# Autodesk Inventor assembly: Irradiation Fixture V1
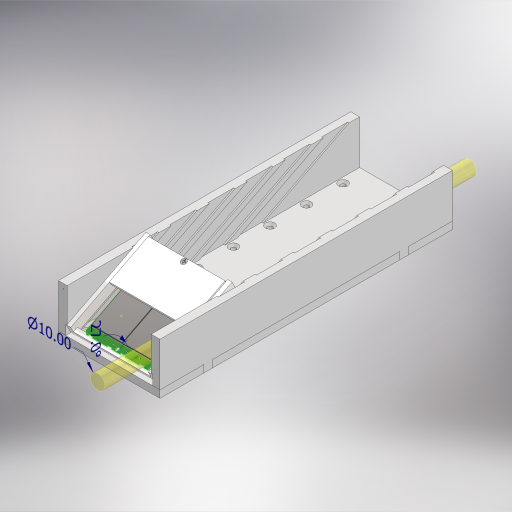
[picture p0: Inventor's stored thumbnail of the model, 512x512]
Saved by Autodesk Inventor 2024 (Build 280153000, 153)
## iProperties
Created: 2024-03-20
Part Number: Irradiation Fixture V1
Document SubType Name: Assembly
Designer: cfang
Author: cfang
## Documents named in this file (4)
- C:\Users\cfang\Desktop\nebraska-silicon-lab\Hardware\ETL\Irradiation Fixture\Irradiation Fixture V1.iam
- C:\Users\cfang\Desktop\nebraska-silicon-lab\Hardware\ETL\Irradiation Fixture\Module Cradle V1.iam
- C:\Users\cfang\Desktop\nebraska-silicon-lab\Hardware\ETL\Irradiation Fixture\Beam Profile.ipt
- C:\Users\cfang\Desktop\nebraska-silicon-lab\Hardware\ETL\Irradiation Fixture\Module with Cover V1.iam
## Components (3 placed, 3 different names)
1. Module Cradle V1:1 [sub-assembly] — Angle:1
2. Beam Profile:1 — Angle:1
3. Module with Cover V1:1 [sub-assembly]
## Relationships (3: Mate 2, Angle 1)
- [Mate]: Module Cradle V1:1 ↔ Module with Cover V1:1
- Angle:1 (0 deg): Module Cradle V1:1 ↔ Beam Profile:1
- [Mate]: Module Cradle V1:1 ↔ Module with Cover V1:1
